# Autodesk Inventor assembly: robot4
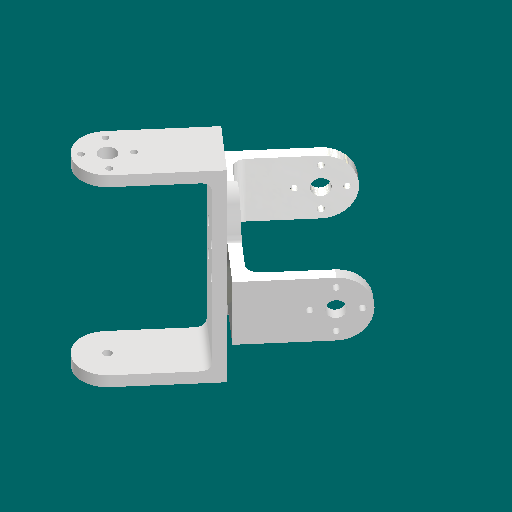
[picture p0: Inventor's stored thumbnail of the model, 512x512]
Saved by Autodesk Inventor 2026.1 (Build 301233000, 233)
## iProperties
Created: 2025-11-03
Part Number: robot4
Document SubType Name: Assembly
Designer: emanuel
Author: emanuel
## Documents named in this file (3)
- C:\Users\emanuel\UnFolder\SpiderRobo\3dmodel\coxa.iam
- C:\Users\emanuel\UnFolder\SpiderRobo\3dmodel\C1.ipt
- C:\Users\emanuel\UnFolder\SpiderRobo\3dmodel\C2.ipt
## Components (2 placed, 2 different names)
1. C2:2 — Mate:130, Mate:131, Mate:132, Mate:133, Mate:134
2. C1:1 — Mate:130, Mate:131, Mate:132, Mate:133, Mate:134
## Relationships (5: Mate 5)
- Mate:130: C2:2 ↔ C1:1
- Mate:131: C2:2 ↔ C1:1
- Mate:132: C2:2 ↔ C1:1
- Mate:133: C2:2 ↔ C1:1
- Mate:134: C2:2 ↔ C1:1
